# Autodesk Inventor assembly: CP2x2
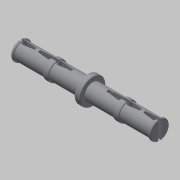
[picture p0: Inventor's stored thumbnail of the model, 180x180]
Saved by Autodesk Inventor 2019.3 (Build 233278000, 278)
## iProperties
Created: 2019-02-05
Part Number: CP2x2
Document SubType Name: Assembly
Designer: Varga Daniel
Author: Varga Daniel
## Documents named in this file (6)
- C:\!_Dani\!_cloud\OneDrive\!_munka\Revolution\RevvyDemoKit\Structural parts\Connetor Pins\CP1+x1+\CP2x2.iam
- C:\!_Dani\!_cloud\OneDrive\!_munka\Revolution\RevvyDemoKit\Structural parts\Connetor Pins\Connector_pin_collar.ipt
- C:\!_Dani\!_cloud\OneDrive\!_munka\Revolution\RevvyDemoKit\Structural parts\Connetor Pins\Connector_pin_stick.ipt
- C:\!_Dani\!_cloud\OneDrive\!_munka\Revolution\RevvyDemoKit\Structural parts\Connetor Pins\Connector_pin_stack_stick.ipt
- C:\!_Dani\!_cloud\OneDrive\!_munka\Revolution\RevvyDemoKit\Structural parts\Connetor Pins\Connector_pin_base.ipt
- C:\!_Dani\!_cloud\OneDrive\!_munka\Revolution\RevvyDemoKit\Structural parts\Connetor Pins\CP1+x1+.iam
## Components (6 placed, 3 different names)
1. Connector_pin_collar:1 — Mate:1, Mate:2, Mate:3, Mate:6, Mate:7
2. Connector_pin_stick:1 — Mate:2, Mate:3, Flush:1, Angle:1, Mate:10, Mate:11, Angle:3
3. Connector_pin_collar:2 — Mate:6, Mate:7
4. Connector_pin_stick:2 — Flush:1, Mate:8, Mate:9, Angle:2
5. Connector_pin_stack_stick:2 — Mate:10, Mate:11, Angle:3
6. Connector_pin_stack_stick:1 — Mate:8, Mate:9, Angle:2
## Component patterns: (1 elements, first: Connector_pin_stack_stick:2), (1 elements, first: Connector_pin_stack_stick:1)
## Relationships (15: Mate 11, Angle 3, Flush 1)
- Mate:1: Connector_pin_collar:1
- Mate:2: Connector_pin_collar:1 ↔ Connector_pin_stick:1
- Mate:3: Connector_pin_collar:1 ↔ Connector_pin_stick:1
- [Mate]: Connector_pin_collar:2 ↔ Connector_pin_stick:2
- [Mate]: Connector_pin_collar:2 ↔ Connector_pin_stick:2
- Mate:6: Connector_pin_collar:1 ↔ Connector_pin_collar:2
- Mate:7: Connector_pin_collar:1 ↔ Connector_pin_collar:2
- Flush:1: Connector_pin_stick:1 ↔ Connector_pin_stick:2
- Angle:1 (0 deg): Connector_pin_stick:1
- Mate:8: Connector_pin_stick:2 ↔ Connector_pin_stack_stick:1
- Mate:9: Connector_pin_stick:2 ↔ Connector_pin_stack_stick:1
- Angle:2 (0 deg): Connector_pin_stick:2 ↔ Connector_pin_stack_stick:1
- Mate:10: Connector_pin_stick:1 ↔ Connector_pin_stack_stick:2
- Mate:11: Connector_pin_stick:1 ↔ Connector_pin_stack_stick:2
- Angle:3 (0 deg): Connector_pin_stick:1 ↔ Connector_pin_stack_stick:2
## Named parameters: d3_d1 = 0 mm, d4_d2 = 0 mm, Collar_thickness = 1.7 mm, Pin_diameter = 4.875 mm, Collar_diameter = 7.5 mm, Pin_overall_length = 20 mm, Pin_inner_length = 8.5 mm, Upper_ring_diameter = 5.5 mm, Upper_ring_thickness = 0.7 mm, Pin_stack_height = 10.2 mm, Stack_num_left = 1, Stack_num_right = 1, Inner_pin_diameter = 5.45 mm, Inner_pin_diameter_correction = 0.05 mm
